# Autodesk Inventor assembly: Screen assembly
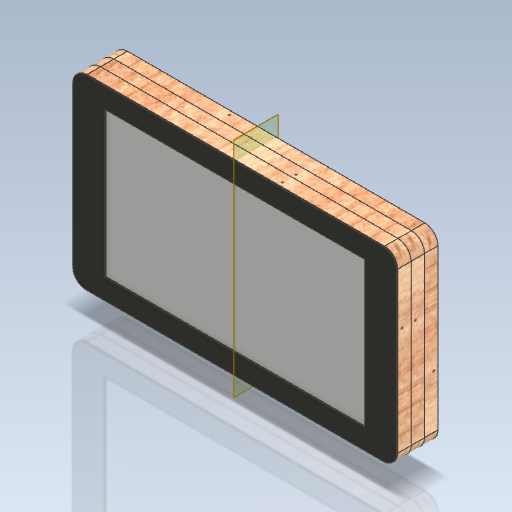
[picture p0: Inventor's stored thumbnail of the model, 512x512]
Saved by Autodesk Inventor 2020.2 (Build 242310000, 310)
## iProperties
Created: 2017-01-12
Part Number: Screen assembly
Document SubType Name: Assembly
Designer: Stefan de Kraker
Title: C:\Users\Stanley\Documents\Inventor\Projects\3D-Printer\3D_Printer_Parts\Selfmade_Parts\Raspberrypi 7inch display\Screen assembly.step
Author: Stanley
## Documents named in this file (6)
- D:\Inventor\Project PAD\LCD\Screen assembly.iam
- D:\Inventor\Project PAD\LCD\Display Lens.ipt
- D:\Inventor\Project PAD\LCD\Display Controller.ipt
- D:\Inventor\Project PAD\LCD\Pi Foundation Display Driver Board.ipt
- D:\Inventor\Project FYS\lcd mount.ipt
- D:\Inventor\Project FYS\lcd mount nut.ipt
## Components (6 placed, 5 different names)
1. Display Lens:1 — Flush:1, Flush:2, Mate:1, Mate:8, Mate:9, Mate:10
2. Display Controller:1 — Flush:1, Flush:2, Mate:1, Mate:2, Mate:3, Mate:4
3. Pi Foundation Display Driver Board:1 — Mate:2, Mate:3, Mate:4
4. lcd mount:1 — Mate:5, Mate:6, Mate:7, Mate:11, Mate:12, Mate:13
5. lcd mount:2 — Mate:5, Mate:6, Mate:7, Mate:8, Mate:9, Mate:10, Symmetry:1
6. lcd mount nut:1 — Mate:11, Mate:12, Mate:13, Symmetry:1
## Relationships (16: Mate 13, Flush 2, Symmetry 1)
- Flush:1 (3.53 mm): Display Lens:1 ↔ Display Controller:1
- Flush:2 (12 mm): Display Lens:1 ↔ Display Controller:1
- Mate:1: Display Lens:1 ↔ Display Controller:1
- Mate:2: Display Controller:1 ↔ Pi Foundation Display Driver Board:1
- Mate:3: Display Controller:1 ↔ Pi Foundation Display Driver Board:1
- Mate:4: Display Controller:1 ↔ Pi Foundation Display Driver Board:1
- Mate:5: lcd mount:1 ↔ lcd mount:2
- Mate:6: lcd mount:1 ↔ lcd mount:2
- Mate:7: lcd mount:1 ↔ lcd mount:2
- Mate:8: Display Lens:1 ↔ lcd mount:2
- Mate:9: Display Lens:1 ↔ lcd mount:2
- Mate:10: Display Lens:1 ↔ lcd mount:2
- Mate:11: lcd mount:1 ↔ lcd mount nut:1
- Mate:12: lcd mount:1 ↔ lcd mount nut:1
- Mate:13: lcd mount:1 ↔ lcd mount nut:1
- Symmetry:1: lcd mount:2 ↔ lcd mount nut:1
